# Autodesk Inventor assembly: 長穴減速_ホーン_2
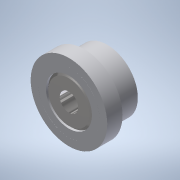
[picture p0: Inventor's stored thumbnail of the model, 180x180]
Saved by Autodesk Inventor 2020 (Build 240168000, 168)
## iProperties
Created: 2016-08-26
Part Number: 長穴減速_ホーン_2
Material: 一般
Document SubType Name: Assembly
Designer: hiro
Author: hiro
## Documents named in this file (4)
- C:\Inventor\OpenPlatform_ver3_0\下半身_160823\リンク\長穴減速_ホーン_2.iam
- C:\Inventor\OpenPlatform_ver3_0\既製品\新規購入\ARU-305_5.ipt
- C:\Inventor\OpenPlatform_ver3_0\既製品\PACK-WSJJ8-6-5.ipt
- C:\Inventor\OpenPlatform_ver3_0\既製品\PACK-WSJJ10-8-2.ipt
## Components (3 placed, 3 different names)
1. ARU-305_5:1 — メイト:1, メイト:2
2. PACK-WSJJ8-6-5:1 — メイト:1, メイト:2, メイト:3, メイト:4
3. PACK-WSJJ10-8-2:1 — メイト:3, メイト:4
## Relationships (4: Mate 4)
- メイト:1 [Mate]: ARU-305_5:1 ↔ PACK-WSJJ8-6-5:1
- メイト:2 [Mate]: ARU-305_5:1 ↔ PACK-WSJJ8-6-5:1
- メイト:3 [Mate]: PACK-WSJJ8-6-5:1 ↔ PACK-WSJJ10-8-2:1
- メイト:4 [Mate]: PACK-WSJJ8-6-5:1 ↔ PACK-WSJJ10-8-2:1
